# Autodesk Inventor assembly: Motor Assembly
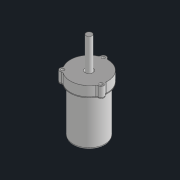
[picture p0: Inventor's stored thumbnail of the model, 180x180]
Saved by Autodesk Inventor 2021 (Build 250183000, 183)
## iProperties
Created: 2020-10-18
Part Number: Motor Assembly
Document SubType Name: Assembly
Designer: Eugene Tang
Mass: 717.382 g
Surface Area: 1406.34 cm^2
Volume: 717.382 cm^3
Density: 1 g/cm^3
Author: Eugene Tang
## Documents named in this file (4)
- C:\Users\teuge\OneDrive - Curtin University of Technology Australia\Y4S2\DFM\Group Project\CAD\Parts\Motor Assembly.iam
- C:\Users\teuge\OneDrive - Curtin University of Technology Australia\Y4S2\DFM\Group Project\CAD\Parts\Motor Pin.ipt
- C:\Users\teuge\OneDrive - Curtin University of Technology Australia\Y4S2\DFM\Group Project\CAD\Parts\Motor Spacer.ipt
- C:\Users\teuge\OneDrive - Curtin University of Technology Australia\Y4S2\DFM\Group Project\CAD\Parts\Motor Cover.ipt
## Components (3 placed, 3 different names)
1. Motor Pin:1 — Mate:1, Mate:2, Mate:3
2. Motor Spacer:1 — Mate:1, Mate:2, Mate:4, Mate:5
3. Motor Cover:1 — Mate:3, Mate:4, Mate:5
## Relationships (5: Mate 5)
- Mate:1: Motor Pin:1 ↔ Motor Spacer:1
- Mate:2: Motor Pin:1 ↔ Motor Spacer:1
- Mate:3: Motor Pin:1 ↔ Motor Cover:1
- Mate:4: Motor Spacer:1 ↔ Motor Cover:1
- Mate:5: Motor Spacer:1 ↔ Motor Cover:1
